# Autodesk Inventor assembly: case
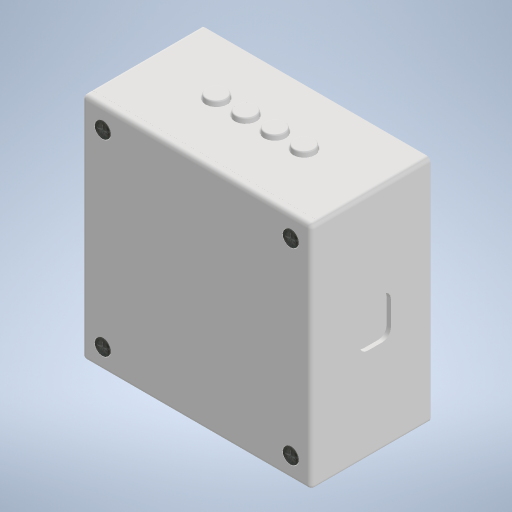
[picture p0: Inventor's stored thumbnail of the model, 512x512]
Saved by Autodesk Inventor 2024 (Build 280153000, 153)
## iProperties
Created: 2023-05-04
Part Number: case
Document SubType Name: Assembly
Designer: cocqu
Author: cocqu
## Documents named in this file (6)
- C:\Projects\sem2\projectwerk\low-voltage-UPS\case\inventor\case.iam
- C:\Projects\sem2\projectwerk\low-voltage-UPS\case\inventor\Base.ipt
- C:\Projects\sem2\projectwerk\low-voltage-UPS\case\inventor\Lid.ipt
- C:\Users\cocqu\Documents\Inventor\Content Center Files\R2024\en-US\ISO 7046-2 H\ISO 7046-2 H - M3.5x5 - 8.8 - H1.ipt
- C:\Projects\sem2\projectwerk\low-voltage-UPS\case\inventor\Button.ipt
- C:\Projects\sem2\projectwerk\low-voltage-UPS\case\inventor\PCB.ipt
## Components (11 placed, 5 different names)
1. Base:1 — Mate:1, Flush:1, Flush:2, Mate:6, Mate:7, Mate:8, Mate:9, Mate:10, Mate:11, Mate:12, Mate:13, Mate:14
2. Lid:1 — Mate:1, Flush:1, Flush:2, Mate:2, Mate:3, Mate:4, Mate:5
3. ISO 7046-2 H M3.5x5 - 8.8 - H1:1 — Mate:2
4. ISO 7046-2 H M3.5x5 - 8.8 - H1:2 — Mate:3
5. ISO 7046-2 H M3.5x5 - 8.8 - H1:3 — Mate:4
6. ISO 7046-2 H M3.5x5 - 8.8 - H1:4 — Mate:5
7. Button:1 — Mate:12, Mate:13
8. Button:2 — Mate:10, Mate:11
9. Button:3 — Mate:8, Mate:9
10. Button:4 — Mate:6, Mate:7
11. PCB:1 — Mate:14
## Relationships (16: Mate 14, Flush 2)
- Mate:1: Base:1 ↔ Lid:1
- Flush:1: Base:1 ↔ Lid:1
- Flush:2: Base:1 ↔ Lid:1
- Mate:2: Lid:1 ↔ ISO 7046-2 H M3.5x5 - 8.8 - H1:1
- Mate:3: Lid:1 ↔ ISO 7046-2 H M3.5x5 - 8.8 - H1:2
- Mate:4: Lid:1 ↔ ISO 7046-2 H M3.5x5 - 8.8 - H1:3
- Mate:5: Lid:1 ↔ ISO 7046-2 H M3.5x5 - 8.8 - H1:4
- Mate:6: Base:1 ↔ Button:4
- Mate:7: Base:1 ↔ Button:4
- Mate:8: Base:1 ↔ Button:3
- Mate:9: Base:1 ↔ Button:3
- Mate:10: Base:1 ↔ Button:2
- Mate:11: Base:1 ↔ Button:2
- Mate:12: Base:1 ↔ Button:1
- Mate:13: Base:1 ↔ Button:1
- Mate:14: Base:1 ↔ PCB:1
